# Autodesk Inventor assembly: s-assy-shooter_motor
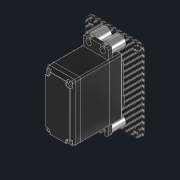
[picture p0: Inventor's stored thumbnail of the model, 180x180]
Saved by Autodesk Inventor 2022 (Build 260153000, 153)
## iProperties
Created: 2021-08-27
Part Number: s-assy-shooter_motor
Document SubType Name: Assembly
Designer: Yuta Kage
Author: Yuta Kage
## Documents named in this file (4)
- C:\Users\yuta0\Documents\GitHub\catchrobo_hardware\assy-shooter\s-assy-shooter_motor.iam
- C:\Users\yuta0\Documents\GitHub\catchrobo_hardware\assy-robot\MG_996R.iam
- C:\Users\yuta0\Documents\GitHub\catchrobo_hardware\assy-shooter\s_carbon_plate4.ipt
- C:\Users\yuta0\Documents\GitHub\catchrobo_hardware\assy-robot\ARF-410E.ipt
## Components (6 placed, 3 different names)
1. MG_996R:1 [sub-assembly] — メイト:18, メイト:19, メイト:20, メイト:22, メイト:24, メイト:25, メイト:35
2. s_carbon_plate4:1 — メイト:18, メイト:19, メイト:20, メイト:23, メイト:33, メイト:34, メイト:36
3. ARF-410E:2 — メイト:22, メイト:23
4. ARF-410E:3 — メイト:24, メイト:25
5. ARF-410E:4 — メイト:33, メイト:34
6. ARF-410E:5 — メイト:35, メイト:36
## Relationships (11: Mate 11)
- メイト:18 [Mate]: MG_996R:1 ↔ s_carbon_plate4:1
- メイト:19 [Mate]: MG_996R:1 ↔ s_carbon_plate4:1
- メイト:20 [Mate] (10 mm): MG_996R:1 ↔ s_carbon_plate4:1
- メイト:22 [Mate]: MG_996R:1 ↔ ARF-410E:2
- メイト:23 [Mate]: s_carbon_plate4:1 ↔ ARF-410E:2
- メイト:24 [Mate]: MG_996R:1 ↔ ARF-410E:3
- メイト:25 [Mate]: MG_996R:1 ↔ ARF-410E:3
- メイト:33 [Mate]: s_carbon_plate4:1 ↔ ARF-410E:4
- メイト:34 [Mate]: s_carbon_plate4:1 ↔ ARF-410E:4
- メイト:35 [Mate]: MG_996R:1 ↔ ARF-410E:5
- メイト:36 [Mate]: s_carbon_plate4:1 ↔ ARF-410E:5
